# Autodesk Inventor assembly: Swing_Arm_03
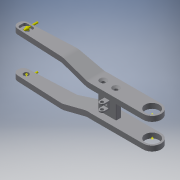
[picture p0: Inventor's stored thumbnail of the model, 180x180]
Saved by Autodesk Inventor 2016 (Build 200138000, 138)
## iProperties
Created: 2016-02-09
Part Number: Swing_Arm_03
Document SubType Name: Assembly
Designer: nils
Author: nils
## Documents named in this file (10)
- D:\bikair\Bikair_CAD-1\Source\Rear_Train\Swing_Arm_03.iam
- D:\bikair\Bikair_CAD-1\Source\Rear_Train\Profile_Straight_03.ipt
- D:\bikair\Bikair_CAD-1\Source\Rear_Train\Profile_Middle_03.ipt
- D:\bikair\Bikair_CAD-1\Source\Rear_Train\Damper_Mount_03.ipt
- D:\bikair\Bikair_CAD-1\Source\Rear_Train\Swing_Arm_03\AIP\FEA\boqvtipog.fins
- D:\bikair\Bikair_CAD-1\Source\Rear_Train\Swing_Arm_03\AIP\FEA\boqvtiqcg.fsat
- D:\bikair\Bikair_CAD-1\Source\Rear_Train\Swing_Arm_03\AIP\FEA\boqvtiqe8.ftes
- D:\bikair\Bikair_CAD-1\Source\Rear_Train\Swing_Arm_03\AIP\FEA\boqvtiqio.fwiz
- D:\bikair\Bikair_CAD-1\Source\Rear_Train\Swing_Arm_03\AIP\FEA\boqvtirq8.fmsh
- D:\bikair\Bikair_CAD-1\Source\Rear_Train\Swing_Arm_03\AIP\FEA\boqvtirr4.fres
## Components (4 placed, 3 different names)
1. Profile_Straight_03:1 — Mate:1, Mate:3, Mate:4
2. Profile_Straight_03:2 — Mate:2, Mate:5, Mate:6, Angle:1
3. Profile_Middle_03:1 — Mate:1, Mate:2, Mate:3, Mate:4, Mate:5, Mate:6, Mate:7, Mate:8
4. Damper_Mount_03:1 — Mate:7, Angle:1, Mate:8
## Relationships (9: Mate 8, Angle 1)
- Mate:1: Profile_Straight_03:1 ↔ Profile_Middle_03:1
- Mate:2: Profile_Straight_03:2 ↔ Profile_Middle_03:1
- Mate:3: Profile_Straight_03:1 ↔ Profile_Middle_03:1
- Mate:4: Profile_Straight_03:1 ↔ Profile_Middle_03:1
- Mate:5: Profile_Straight_03:2 ↔ Profile_Middle_03:1
- Mate:6: Profile_Straight_03:2 ↔ Profile_Middle_03:1
- Mate:7: Profile_Middle_03:1 ↔ Damper_Mount_03:1
- Angle:1 (0 deg): Profile_Straight_03:2 ↔ Damper_Mount_03:1
- Mate:8: Profile_Middle_03:1 ↔ Damper_Mount_03:1
## Named parameters: sa_0 = -1.8607e-09, sa_1 = -400000, sa_2 = -1.127e-10, sa_3 = -1.1224e-09, sa_4 = -400000, sa_5 = -1.127e-10
note: some values were not read from the file. Shown as the stored number, unit unknown: "sa_0", "sa_1", "sa_2", "sa_3", "sa_4", "sa_5".
